# Autodesk Inventor assembly: Robot
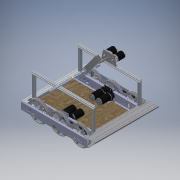
[picture p0: Inventor's stored thumbnail of the model, 180x180]
Saved by Autodesk Inventor 2016 (Build 200138000, 138)
## iProperties
Created: 2016-01-27
Part Number: Robot
Document SubType Name: Assembly
Designer: PrashantBIA
Author: PrashantBIA
## Documents named in this file (22)
- C:\Users\Andrew\Documents\GitHub\2016RobotCADFiles\Robot.iam
- C:\Users\Andrew\Documents\GitHub\2016RobotCADFiles\Drive Train\AM14U3+Square+REV1-1.iam
- C:\Users\Andrew\Documents\GitHub\2016RobotCADFiles\Electronic Parts\CIM Motor.ipt
- C:\Users\Andrew\Documents\GitHub\2016RobotCADFiles\1x1\22in.ipt
- C:\Users\Andrew\Documents\GitHub\2016RobotCADFiles\Electronic Parts\Electrical Board Assembly.iam
- C:\Users\Andrew\Documents\GitHub\2016RobotCADFiles\Electronic Parts\am-2939+BatteryHolder.ipt
- C:\Users\Andrew\Documents\GitHub\2016RobotCADFiles\Electronic Parts\ELEC_Battery_NP18-12B.ipt
- C:\Users\Andrew\Documents\GitHub\2016RobotCADFiles\Special Assemblies\8inWheel.iam
- C:\Users\Andrew\Documents\GitHub\2016RobotCADFiles\Special Assemblies\Middle8inWheel.iam
- C:\Users\Andrew\Documents\GitHub\2016RobotCADFiles\Drive Train\am-3356_AM14U3_End_Sheet_Wedge (1).ipt
- C:\Users\Andrew\Documents\GitHub\2016RobotCADFiles\Drive Train\skid plate.ipt
- C:\Users\Andrew\Documents\GitHub\2016RobotCADFiles\Kicker\short rev x wing.ipt
- C:\Users\Andrew\Documents\GitHub\2016RobotCADFiles\Kicker\long rev x wing.ipt
- C:\Users\Andrew\Documents\GitHub\2016RobotCADFiles\Kicker\CIMple Box.ipt
- C:\Users\Andrew\Documents\GitHub\2016RobotCADFiles\Drive Train\TB Output Shaft Hex L-Base 2.ipt
- C:\Users\Andrew\Documents\GitHub\2016RobotCADFiles\Kicker\10inshaft.ipt
- C:\Users\Andrew\Documents\GitHub\2016RobotCADFiles\Kicker\217-4008-STEP-20140807.ipt
- C:\Users\Andrew\Documents\GitHub\2016RobotCADFiles\Kicker\11in.ipt
- C:\Users\Andrew\Documents\GitHub\2016RobotCADFiles\Shooter\am-0096a+500+Hex+Hub+r2.ipt
- C:\Users\Andrew\Documents\GitHub\2016RobotCADFiles\Shooter\miniCIM.ipt
- C:\Users\Andrew\Documents\GitHub\2016RobotCADFiles\Kicker\10inshaft - Copy.ipt
- C:\Users\Andrew\Documents\GitHub\2016RobotCADFiles\Kicker\217-2737.20121205.ipt
## Components (35 placed, 21 different names)
1. short rev x wing:1 — Mate:50, Mate:54, Flush:7, Mate:57, Flush:8, Flush:9
2. short rev x wing:2 — Mate:51, Flush:5, Mate:52, Flush:6, Mate:53
3. short rev x wing:3 — Mate:48, Mate:56, Mate:58
4. short rev x wing:4 — Mate:49, Mate:55, Flush:10, Flush:11
5. long rev x wing:1 — Flush:5, Mate:52, Flush:6, Mate:58
6. long rev x wing:2 — Mate:57, Flush:8, Flush:9, Flush:10, Flush:11, Mate:59, Flush:12, Flush:14
7. CIMple Box:1 — Mate:59, Flush:12, Flush:14, Mate:60, Flush:15, Mate:69, Mate:70, Mate:71, Mate:72
8. TB Output Shaft Hex L-Base 2:1 — Mate:60, Flush:15, Mate:61, Flush:16, Flush:17, Mate:62
9. 10inshaft:1 — Mate:61, Flush:16, Flush:17, Flush:18, Flush:19, Mate:66, Mate:67, Flush:22, Mate:73, Flush:23, Mate:75, Mate:76, Mate:78, Mate:79
10. 217-4008-STEP-20140807:1 — Flush:18, Mate:62, Flush:19
11. 11in:1 — Mate:63, Mate:64, Mate:65, Flush:20, Flush:21, Mate:77
12. am-0096a+500+Hex+Hub+r2:1 — Mate:63, Mate:64, Mate:65, Flush:20, Mate:66, Mate:67, Mate:74
13. miniCIM:1 — Mate:71, Mate:72
14. miniCIM:2 — Mate:69, Mate:70
15. 10inshaft - Copy:1 — Flush:22, Mate:73, Flush:23
16. 217-2737.20121205:1 — Mate:74, Mate:75, Mate:76
17. 217-2737.20121205:2 — Mate:77, Mate:78, Mate:79
18. skid plate:1 — Mate:45, Mate:46, Mate:47
19. am-3356_AM14U3_End_Sheet_Wedge (1):1 — Mate:42, Mate:43, Mate:44, Mate:50, Mate:53, Mate:54, Flush:7
20. CIM Motor:4 — Insert:2
21. CIM Motor:3 — Insert:1
22. CIM Motor:2 — Insert:3
23. CIM Motor:1 — Insert:4
24. AM14U3+Square+REV1-1:1 [sub-assembly] — Insert:1, Insert:2, Flush:1, Mate:15, Mate:16, Flush:2, Mate:19, Mate:20, Mate:21, Mate:24, Mate:25, Mate:26, Mate:27, Mate:28, Mate:30, Mate:31, Mate:32, Mate:33, Mate:35, Mate:36, Mate:38, Insert:3, Insert:4, Mate:39, Mate:40, Mate:41, Mate:42, Mate:43, Mate:44, Mate:45, Mate:46, Mate:47, Mate:48, Mate:49, Mate:51, Mate:55, Mate:56, Flush:21
25. 22in:1 — Flush:1, Mate:15, Mate:17, Flush:4
26. 22in:2 — Mate:16, Flush:2, Mate:17, Flush:3, Mate:18
27. Electrical Board Assembly:1 [sub-assembly] — Flush:3, Mate:18, Flush:4
28. am-2939+BatteryHolder:1 — Mate:19, Mate:20, Mate:21, Mate:22, Mate:23
29. ELEC_Battery_NP18-12B:1 — Mate:22, Mate:23, Mate:24
30. Middle8inWheel:2 [sub-assembly] — Mate:36, Mate:39
31. Middle8inWheel:1 [sub-assembly] — Mate:35, Mate:38
32. 8inWheel:4 [sub-assembly] — Mate:28, Mate:41
33. 8inWheel:3 [sub-assembly] — Mate:32, Mate:33, Mate:40
34. 8inWheel:2 [sub-assembly] — Mate:30, Mate:31
35. 8inWheel:1 [sub-assembly] — Mate:25, Mate:26, Mate:27
## Relationships (87: Mate 61, Flush 22, Insert 4)
- Insert:1: CIM Motor:3 ↔ AM14U3+Square+REV1-1:1
- Insert:2: CIM Motor:4 ↔ AM14U3+Square+REV1-1:1
- Flush:1: AM14U3+Square+REV1-1:1 ↔ 22in:1
- Mate:15: AM14U3+Square+REV1-1:1 ↔ 22in:1
- Mate:16: AM14U3+Square+REV1-1:1 ↔ 22in:2
- Flush:2: AM14U3+Square+REV1-1:1 ↔ 22in:2
- Mate:17 (304.8 mm): 22in:1 ↔ 22in:2
- Flush:3: 22in:2 ↔ Electrical Board Assembly:1
- Mate:18: 22in:2 ↔ Electrical Board Assembly:1
- Flush:4 (-76.2 mm): 22in:1 ↔ Electrical Board Assembly:1
- Mate:19: AM14U3+Square+REV1-1:1 ↔ am-2939+BatteryHolder:1
- Mate:20: AM14U3+Square+REV1-1:1 ↔ am-2939+BatteryHolder:1
- Mate:21: AM14U3+Square+REV1-1:1 ↔ am-2939+BatteryHolder:1
- Mate:22: am-2939+BatteryHolder:1 ↔ ELEC_Battery_NP18-12B:1
- Mate:23: am-2939+BatteryHolder:1 ↔ ELEC_Battery_NP18-12B:1
- Mate:24: AM14U3+Square+REV1-1:1 ↔ ELEC_Battery_NP18-12B:1
- Mate:25: AM14U3+Square+REV1-1:1 ↔ 8inWheel:1
- Mate:26: AM14U3+Square+REV1-1:1 ↔ 8inWheel:1
- Mate:27: AM14U3+Square+REV1-1:1 ↔ 8inWheel:1
- Mate:28: AM14U3+Square+REV1-1:1 ↔ 8inWheel:4
- Mate:30: AM14U3+Square+REV1-1:1 ↔ 8inWheel:2
- Mate:31: AM14U3+Square+REV1-1:1 ↔ 8inWheel:2
- Mate:32: AM14U3+Square+REV1-1:1 ↔ 8inWheel:3
- Mate:33: AM14U3+Square+REV1-1:1 ↔ 8inWheel:3
- Mate:35: AM14U3+Square+REV1-1:1 ↔ Middle8inWheel:1
- Mate:36: AM14U3+Square+REV1-1:1 ↔ Middle8inWheel:2
- Mate:38: AM14U3+Square+REV1-1:1 ↔ Middle8inWheel:1
- Insert:3: CIM Motor:2 ↔ AM14U3+Square+REV1-1:1
- Insert:4: CIM Motor:1 ↔ AM14U3+Square+REV1-1:1
- Mate:39: AM14U3+Square+REV1-1:1 ↔ Middle8inWheel:2
- Mate:40: AM14U3+Square+REV1-1:1 ↔ 8inWheel:3
- Mate:41: AM14U3+Square+REV1-1:1 ↔ 8inWheel:4
- Mate:42: am-3356_AM14U3_End_Sheet_Wedge (1):1 ↔ AM14U3+Square+REV1-1:1
- Mate:43: am-3356_AM14U3_End_Sheet_Wedge (1):1 ↔ AM14U3+Square+REV1-1:1
- Mate:44: am-3356_AM14U3_End_Sheet_Wedge (1):1 ↔ AM14U3+Square+REV1-1:1
- Mate:45: skid plate:1 ↔ AM14U3+Square+REV1-1:1
- Mate:46: skid plate:1 ↔ AM14U3+Square+REV1-1:1
- Mate:47: skid plate:1 ↔ AM14U3+Square+REV1-1:1
- Mate:48: short rev x wing:3 ↔ AM14U3+Square+REV1-1:1
- Mate:49: short rev x wing:4 ↔ AM14U3+Square+REV1-1:1
- Mate:50: short rev x wing:1 ↔ am-3356_AM14U3_End_Sheet_Wedge (1):1
- Mate:51: short rev x wing:2 ↔ AM14U3+Square+REV1-1:1
- Flush:5: short rev x wing:2 ↔ long rev x wing:1
- Mate:52: short rev x wing:2 ↔ long rev x wing:1
- Flush:6: short rev x wing:2 ↔ long rev x wing:1
- Mate:53: short rev x wing:2 ↔ am-3356_AM14U3_End_Sheet_Wedge (1):1
- Mate:54: short rev x wing:1 ↔ am-3356_AM14U3_End_Sheet_Wedge (1):1
- Mate:55: short rev x wing:4 ↔ AM14U3+Square+REV1-1:1
- Mate:56: short rev x wing:3 ↔ AM14U3+Square+REV1-1:1
- Flush:7: short rev x wing:1 ↔ am-3356_AM14U3_End_Sheet_Wedge (1):1
- Mate:57: short rev x wing:1 ↔ long rev x wing:2
- Flush:8: short rev x wing:1 ↔ long rev x wing:2
- Flush:9: short rev x wing:1 ↔ long rev x wing:2
- Mate:58: short rev x wing:3 ↔ long rev x wing:1
- Flush:10: short rev x wing:4 ↔ long rev x wing:2
- Flush:11: short rev x wing:4 ↔ long rev x wing:2
- Mate:59: long rev x wing:2 ↔ CIMple Box:1
- Flush:12: long rev x wing:2 ↔ CIMple Box:1
- Flush:14 (252.4125 mm): long rev x wing:2 ↔ CIMple Box:1
- Mate:60: CIMple Box:1 ↔ TB Output Shaft Hex L-Base 2:1
- Flush:15 (-12.7 mm): CIMple Box:1 ↔ TB Output Shaft Hex L-Base 2:1
- Mate:61: TB Output Shaft Hex L-Base 2:1 ↔ 10inshaft:1
- Flush:16: TB Output Shaft Hex L-Base 2:1 ↔ 10inshaft:1
- Flush:17: TB Output Shaft Hex L-Base 2:1 ↔ 10inshaft:1
- Flush:18: 10inshaft:1 ↔ 217-4008-STEP-20140807:1
- Mate:62: TB Output Shaft Hex L-Base 2:1 ↔ 217-4008-STEP-20140807:1
- Flush:19 (-19.05 mm): 10inshaft:1 ↔ 217-4008-STEP-20140807:1
- Mate:63: 11in:1 ↔ am-0096a+500+Hex+Hub+r2:1
- Mate:64 (-25.4 mm): 11in:1 ↔ am-0096a+500+Hex+Hub+r2:1
- Mate:65 (-25.4 mm): 11in:1 ↔ am-0096a+500+Hex+Hub+r2:1
- Flush:20 (44.45 mm): 11in:1 ↔ am-0096a+500+Hex+Hub+r2:1
- Mate:66: 10inshaft:1 ↔ am-0096a+500+Hex+Hub+r2:1
- Mate:67: 10inshaft:1 ↔ am-0096a+500+Hex+Hub+r2:1
- Mate:69: CIMple Box:1 ↔ miniCIM:2
- Mate:70: CIMple Box:1 ↔ miniCIM:2
- Mate:71: CIMple Box:1 ↔ miniCIM:1
- Mate:72: CIMple Box:1 ↔ miniCIM:1
- Flush:21 (349.25 mm): 11in:1 ↔ AM14U3+Square+REV1-1:1
- Flush:22: 10inshaft:1 ↔ 10inshaft - Copy:1
- Mate:73: 10inshaft:1 ↔ 10inshaft - Copy:1
- Flush:23: 10inshaft:1 ↔ 10inshaft - Copy:1
- Mate:74: am-0096a+500+Hex+Hub+r2:1 ↔ 217-2737.20121205:1
- Mate:75: 10inshaft:1 ↔ 217-2737.20121205:1
- Mate:76: 10inshaft:1 ↔ 217-2737.20121205:1
- Mate:77: 11in:1 ↔ 217-2737.20121205:2
- Mate:78: 10inshaft:1 ↔ 217-2737.20121205:2
- Mate:79: 10inshaft:1 ↔ 217-2737.20121205:2
